# Autodesk Inventor assembly: Assembly1
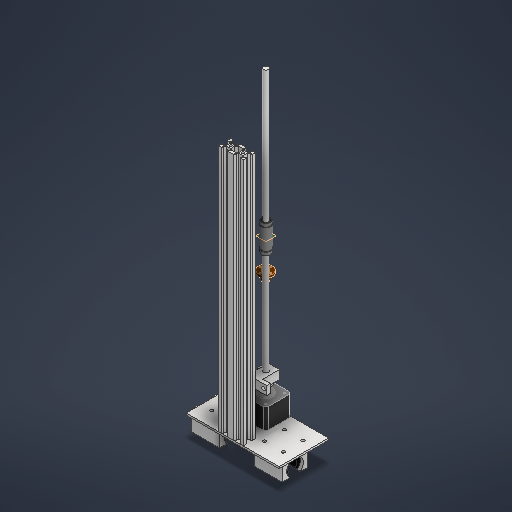
[picture p0: Inventor's stored thumbnail of the model, 512x512]
Saved by Autodesk Inventor 2025.1 (Build 291241000, 241)
## iProperties
Created: 2024-12-18
Part Number: Assembly1
Document SubType Name: Assembly
Designer: jerem
Author: jerem
## Documents named in this file (11)
- C:\Users\jerem\Documents\GitHub\Perovskite-Automated-Synthesis-System\CAD\Gantry\Assembly1.iam
- C:\Users\jerem\Documents\GitHub\Perovskite-Automated-Synthesis-System\CAD\Non 3D Printed Parts\X Axis Base Plate.ipt
- C:\Users\jerem\Documents\GitHub\Perovskite-Automated-Synthesis-System\CAD\Non 3D Printed Parts\Linear Rails\Linear Rail Slider Block.ipt
- C:\Users\jerem\Documents\GitHub\Perovskite-Automated-Synthesis-System\CAD\Non 3D Printed Parts\Extrusion\V Extrustion 40x400mm.ipt
- C:\Users\jerem\Documents\GitHub\Perovskite-Automated-Synthesis-System\CAD\Non 3D Printed Parts\Motors and Servos\NEMA17 Stepper Motor.ipt
- C:\Users\jerem\Documents\GitHub\Perovskite-Automated-Synthesis-System\CAD\Non 3D Printed Parts\Threaded Rod 300mm.ipt
- C:\Users\jerem\Documents\GitHub\Perovskite-Automated-Synthesis-System\CAD\Non 3D Printed Parts\Rod Coupler.ipt
- C:\Users\jerem\Documents\GitHub\Perovskite-Automated-Synthesis-System\CAD\Non 3D Printed Parts\Linear Rails\8mm Linear Rod.ipt
- C:\Users\jerem\Documents\GitHub\Perovskite-Automated-Synthesis-System\CAD\Non 3D Printed Parts\Linear Rails\Linear Rod Holder SK8.ipt
- C:\Users\jerem\Documents\GitHub\Perovskite-Automated-Synthesis-System\CAD\Non 3D Printed Parts\Linear Rails\Linear Bearing 8mm Round.ipt
- C:\Users\jerem\Documents\GitHub\Perovskite-Automated-Synthesis-System\CAD\Non 3D Printed Parts\Leadscrew.ipt
## Components (11 placed, 10 different names)
1. X Axis Base Plate:1 — Mate:5, Mate:6, Mate:7, Mate:8, Flush:1, Flush:2
2. Linear Rail Slider Block:1 — Mate:7
3. Linear Rail Slider Block:2 — Mate:6
4. V Extrustion 40x400mm:1 — Mate:5, Mate:9, Flush:1
5. NEMA17 Stepper Motor:1 — Mate:8, Flush:2
6. Threaded Rod 300mm:1 — Mate:12
7. Rod Coupler:1
8. 8mm Linear Rod:1 — Mate:10, Flush:3, Mate:11
9. Linear Rod Holder SK8:1 — Mate:9, Mate:10, Flush:3
10. Linear Bearing 8mm Round:1 — Mate:11
11. Leadscrew:1 — Mate:12
## Relationships (15: Mate 12, Flush 3)
- [Mate]: NEMA17 Stepper Motor:1 ↔ Rod Coupler:1
- [Mate]: Threaded Rod 300mm:1 ↔ Rod Coupler:1
- [Mate] (-8 mm): NEMA17 Stepper Motor:1 ↔ Rod Coupler:1
- [Mate] (-8 mm): Threaded Rod 300mm:1 ↔ Rod Coupler:1
- Mate:5: X Axis Base Plate:1 ↔ V Extrustion 40x400mm:1
- Mate:6: X Axis Base Plate:1 ↔ Linear Rail Slider Block:2
- Mate:7: X Axis Base Plate:1 ↔ Linear Rail Slider Block:1
- Mate:8: X Axis Base Plate:1 ↔ NEMA17 Stepper Motor:1
- Mate:9: V Extrustion 40x400mm:1 ↔ Linear Rod Holder SK8:1
- Flush:1: X Axis Base Plate:1 ↔ V Extrustion 40x400mm:1
- Flush:2: X Axis Base Plate:1 ↔ NEMA17 Stepper Motor:1
- Mate:10: 8mm Linear Rod:1 ↔ Linear Rod Holder SK8:1
- Flush:3: 8mm Linear Rod:1 ↔ Linear Rod Holder SK8:1
- Mate:11: 8mm Linear Rod:1 ↔ Linear Bearing 8mm Round:1
- Mate:12: Threaded Rod 300mm:1 ↔ Leadscrew:1
